# Autodesk Inventor assembly: Manillar_freno
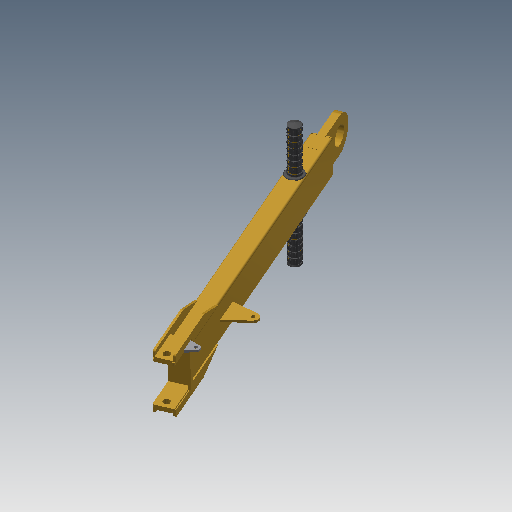
[picture p0: Inventor's stored thumbnail of the model, 512x512]
Saved by Autodesk Inventor 2019 (Build 230136000, 136)
## iProperties
Created: 2020-02-07
Part Number: Manillar_freno
Document SubType Name: Assembly
Designer: Juan Carlos Botero
Author: Juan Carlos Botero
## Documents named in this file (3)
- D:\Drives\OneDrive\Carlos_2\02 TRABAJOS\MULTIPLO\Conveyor\ENSAMBLE\Manillar_freno.iam
- D:\Drives\OneDrive\Carlos_2\02 TRABAJOS\MULTIPLO\Conveyor\ENSAMBLE\Solid2.ipt
- D:\Drives\OneDrive\Carlos_2\02 TRABAJOS\MULTIPLO\Conveyor\ENSAMBLE\manillar tiro.iam
## Components (2 placed, 2 different names)
1. Solid2:1
2. manillar tiro:1 [sub-assembly]
## Relationships (3: Mate 2, Flush 1)
- [Mate]: Solid2:1 ↔ manillar tiro:1
- [Mate] (69.147 mm): Solid2:1 ↔ manillar tiro:1
- [Flush]: Solid2:1 ↔ manillar tiro:1
